# Autodesk Inventor assembly: conceptual assembly
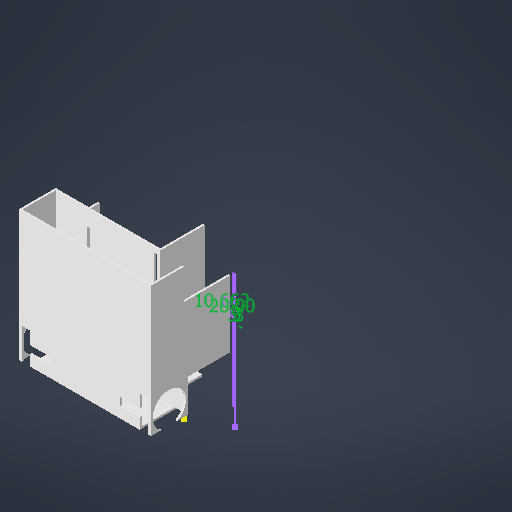
[picture p0: Inventor's stored thumbnail of the model, 512x512]
Saved by Autodesk Inventor 2026.2 (Build 302298000, 298)
## iProperties
Created: 2026-02-03
Part Number: conceptual assembly
Document SubType Name: Assembly
Designer: mones
Author: mones
## Documents named in this file (8)
- C:\Users\small.ab\Desktop\RoboticsGHIT\Unibots_NULondon\hardware\chassis\conceptual assembly.iam
- C:\Users\small.ab\Desktop\RoboticsGHIT\Unibots_NULondon\hardware\chassis\Chassis Conceptual Geo.ipt
- C:\Users\small.ab\Desktop\RoboticsGHIT\Unibots_NULondon\hardware\chassis\inside walls.ipt
- C:\Users\small.ab\Desktop\RoboticsGHIT\Unibots_NULondon\hardware\chassis\lift plate.ipt
- C:\Users\small.ab\Desktop\RoboticsGHIT\Unibots_NULondon\hardware\chassis\inside walls left.ipt
- C:\Users\small.ab\Desktop\RoboticsGHIT\Unibots_NULondon\hardware\chassis\inside walls front.ipt
- C:\Users\small.ab\Downloads\Mecanum Left v5.iam
- C:\Users\small.ab\Downloads\logitech-c920.iam
## Components (7 placed, 7 different names)
1. Chassis Conceptual Geo:1 — Mate:3, Mate:4, Mate:5, Mate:6, Mate:7, Mate:8, Flush:1
2. inside walls:3 — Mate:3, Mate:4, Insert:1, Mate:9
3. lift plate:1 — Insert:1
4. inside walls left:1 — Mate:5, Mate:6, Mate:7
5. inside walls front:1 — Mate:8, Mate:9
6. Mecanum Left v5:1 [sub-assembly] — Flush:1
7. logitech-c920:1 [sub-assembly]
## Relationships (9: Mate 7, Insert 1, Flush 1)
- Mate:3: Chassis Conceptual Geo:1 ↔ inside walls:3
- Mate:4: Chassis Conceptual Geo:1 ↔ inside walls:3
- Insert:1: inside walls:3 ↔ lift plate:1
- Mate:5: Chassis Conceptual Geo:1 ↔ inside walls left:1
- Mate:6: Chassis Conceptual Geo:1 ↔ inside walls left:1
- Mate:7: Chassis Conceptual Geo:1 ↔ inside walls left:1
- Mate:8: Chassis Conceptual Geo:1 ↔ inside walls front:1
- Mate:9: inside walls:3 ↔ inside walls front:1
- Flush:1: Chassis Conceptual Geo:1 ↔ Mecanum Left v5:1
